# Autodesk Inventor assembly: Haus
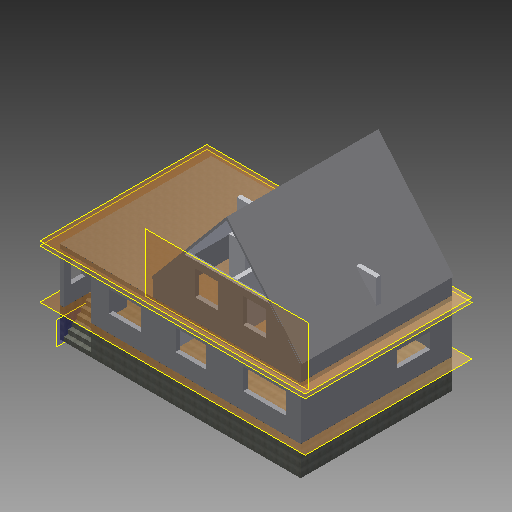
[picture p0: Inventor's stored thumbnail of the model, 512x512]
Saved by Autodesk Inventor 2017 (Build 210142000, 142)
## iProperties
Created: 2017-05-11
Part Number: Haus
Document SubType Name: Assembly
Designer: Fake
Author: Fake
## Documents named in this file (9)
- C:\Users\Fake\Documents\Inventor\Oli_Grundstück\Haus.iam
- C:\Users\Fake\Documents\Inventor\Oli_Grundstück\Grundriss_Haus.ipt
- C:\Users\Fake\Documents\Inventor\Oli_Grundstück\Aussenwand.ipt
- C:\Users\Fake\Documents\Inventor\Oli_Grundstück\Wände_unten.ipt
- C:\Users\Fake\Documents\Inventor\Oli_Grundstück\Zwischendecke.ipt
- C:\Users\Fake\Documents\Inventor\Oli_Grundstück\Wände_oben.ipt
- C:\Users\Fake\Documents\Inventor\Oli_Grundstück\Aussenwände_oben.ipt
- C:\Users\Fake\Documents\Inventor\Oli_Grundstück\Haus_Dach.ipt
- C:\Users\Fake\Documents\Inventor\Oli_Grundstück\Tür.iam
## Components (8 placed, 8 different names)
1. Grundriss_Haus:1 — Fluchtend:1, Fluchtend:2
2. Aussenwand:1 — Fluchtend:1, Fluchtend:3
3. Wände_unten:1 — Fluchtend:2, Passend:1, Passend:2, Passend:3
4. Haus_Dach:1 — Fluchtend:7
5. Tür:1 [sub-assembly] — Passend:1, Passend:2, Passend:3
6. Zwischendecke:1 — Fluchtend:3, Fluchtend:4, Fluchtend:5, Fluchtend:6
7. Wände_oben:1 — Fluchtend:4, Fluchtend:5
8. Aussenwände_oben:1 — Fluchtend:6, Fluchtend:7
## Relationships (10: Flush 7, Mate 3)
- Fluchtend:1 [Flush]: Grundriss_Haus:1 ↔ Aussenwand:1
- Fluchtend:2 [Flush]: Grundriss_Haus:1 ↔ Wände_unten:1
- Fluchtend:3 [Flush]: Aussenwand:1 ↔ Zwischendecke:1
- Fluchtend:4 [Flush]: Zwischendecke:1 ↔ Wände_oben:1
- Fluchtend:5 [Flush]: Zwischendecke:1 ↔ Wände_oben:1
- Fluchtend:6 [Flush]: Zwischendecke:1 ↔ Aussenwände_oben:1
- Fluchtend:7 [Flush]: Haus_Dach:1 ↔ Aussenwände_oben:1
- Passend:1 [Mate]: Wände_unten:1 ↔ Tür:1
- Passend:2 [Mate]: Wände_unten:1 ↔ Tür:1
- Passend:3 [Mate]: Wände_unten:1 ↔ Tür:1
